# Autodesk Inventor assembly: Bar Cabinet Assembly
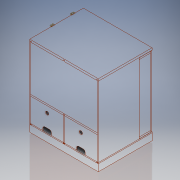
[picture p0: Inventor's stored thumbnail of the model, 180x180]
Saved by Autodesk Inventor 2016 (Build 200138000, 138)
## iProperties
Created: 2017-10-30
Part Number: Bar Cabinet Assembly
Document SubType Name: Assembly
Designer: mathaetaes
Author: mathaetaes
## Documents named in this file (5)
- E:\Projects\3D Printer\printer projects\My Designs\Bar Cabinet\Bar Cabinet Full Assembly.iam
- E:\Projects\3D Printer\printer projects\My Designs\Bar Cabinet\Door.iam
- E:\Projects\3D Printer\printer projects\My Designs\Bar Cabinet\Door 2.iam
- E:\Projects\3D Printer\printer projects\My Designs\Bar Cabinet\Bar Cabinet And Base.iam
- E:\Projects\3D Printer\printer projects\My Designs\Bar Cabinet\Hinge.iam
## Components (5 placed, 4 different names)
1. Bar Cabinet And Base:1 [sub-assembly] — Right Door Hinge, Left Door Hinge, Mate:1, Mate:2, Mate:3, Mate:4, Mate:5, Mate:6
2. Right Door: Door 1 [sub-assembly] — Right Door Hinge
3. Left Door: Door 2 [sub-assembly] — Left Door Hinge
4. Hinge:1 [sub-assembly] — Mate:1, Mate:2, Mate:3
5. Hinge:3 [sub-assembly] — Mate:4, Mate:5, Mate:6
## Relationships (8: Mate 6, RevoluteJoint 2)
- Right Door Hinge [RevoluteJoint]: Bar Cabinet And Base:1 ↔ Right Door: Door 1
- Left Door Hinge [RevoluteJoint]: Bar Cabinet And Base:1 ↔ Left Door: Door 2
- Mate:1: Bar Cabinet And Base:1 ↔ Hinge:1
- Mate:2: Bar Cabinet And Base:1 ↔ Hinge:1
- Mate:3: Bar Cabinet And Base:1 ↔ Hinge:1
- Mate:4: Bar Cabinet And Base:1 ↔ Hinge:3
- Mate:5: Bar Cabinet And Base:1 ↔ Hinge:3
- Mate:6: Bar Cabinet And Base:1 ↔ Hinge:3
